# Autodesk Inventor assembly: mascon-new
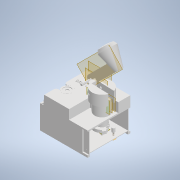
[picture p0: Inventor's stored thumbnail of the model, 180x180]
Saved by Autodesk Inventor 2022 (Build 260153000, 153)
## iProperties
Created: 2021-04-28
Part Number: mascon-new
Document SubType Name: Assembly
Designer: ben
Author: ben
## iProperties of the stored document Pin2.ipt
Created: 2022-01-01
Part Number: Pin2
Material: Steel
Document SubType Name: Modeling
Designer: teh18
Density: 7.85 g/cm^3
Appearance: Default
Author: teh18
## iProperties of the stored document ScrewBase.ipt
Created: 2022-01-01
Part Number: ScrewBase
Material: Steel
Document SubType Name: Modeling
Designer: teh18
Density: 7.85 g/cm^3
Appearance: Default
Author: teh18
## iProperties of the stored document Pin3.ipt
Created: 2022-01-01
Part Number: Pin3
Material: Steel
Document SubType Name: Modeling
Designer: teh18
Density: 7.85 g/cm^3
Appearance: Default
Author: teh18
## iProperties of the stored document Board.ipt
Created: 2022-01-01
Part Number: Board
Material: Steel
Document SubType Name: Modeling
Designer: teh18
Density: 7.85 g/cm^3
Appearance: Default
Author: teh18
## iProperties of the stored document Casing.ipt
Created: 2022-01-01
Part Number: Casing
Material: Steel
Document SubType Name: Modeling
Designer: teh18
Density: 7.85 g/cm^3
Appearance: Default
Author: teh18
## iProperties of the stored document Pin1.ipt
Created: 2022-01-01
Part Number: Pin1
Material: Steel
Document SubType Name: Modeling
Designer: teh18
Density: 7.85 g/cm^3
Appearance: Default
Author: teh18
## iProperties of the stored document PotentiometerB10K.iam
Created: 2020-08-30
Part Number: PotentiometerB10K
Document SubType Name: Assembly
Designer: teh18
Title: D:/OneDrive/Projetos/Yoke FS/V4/PotentiometerToGrabCad/PotentiometerB10K.step
Sending System: Autodesk Translation Framework v9.3.0.1241
Preprocessor: ST-DEVELOPER v18.1
## iProperties of the stored document Shaft.ipt
Created: 2022-01-01
Part Number: Shaft
Material: Steel
Document SubType Name: Modeling
Designer: teh18
Density: 7.85 g/cm^3
Appearance: Default
Author: teh18
## Documents named in this file (20)
- **C:\Users\teh18\Documents\GitHub\r68-bve-mascon\mascon-new.iam*LocalDocs*xAaaaahdaAaaaaaaaAaaaakmpVc*Pin2.ipt
- **C:\Users\teh18\Documents\GitHub\r68-bve-mascon\mascon-new.iam*LocalDocs*xAaaaafdaAaaaaaaaAaaaabwyVb*ScrewBase.ipt
- **C:\Users\teh18\Documents\GitHub\r68-bve-mascon\mascon-new.iam*LocalDocs*xAaaaaccaAaaaaaaaAaaaacpb2b*Pin3.ipt
- **C:\Users\teh18\Documents\GitHub\r68-bve-mascon\mascon-new.iam*LocalDocs*xAaaaagaaAaaaaaaaAaaaqhofGg*Board.ipt
- **C:\Users\teh18\Documents\GitHub\r68-bve-mascon\mascon-new.iam*LocalDocs*xAaaaqjcaAaaaaaaaAaaaat2iJf*Casing.ipt
- **C:\Users\teh18\Documents\GitHub\r68-bve-mascon\mascon-new.iam*LocalDocs*xAaaaqfaaAaaaaaaaAaaaaacoKh*Pin1.ipt
- **C:\Users\teh18\Documents\GitHub\r68-bve-mascon\mascon-new.iam*LocalDocs*xAaaaqhaaAaaaaaaaAaaaaeywJf*PotentiometerB10K.iam
- **C:\Users\teh18\Documents\GitHub\r68-bve-mascon\mascon-new.iam*LocalDocs*xAaaaqrbaAaaaaaaaAaaaalw5Ad*Shaft.ipt
- C:\Users\teh18\Documents\GitHub\r68-bve-mascon\mascon-new.iam
- C:\Users\teh18\Documents\GitHub\r68-bve-mascon\handle\handle.iam
- C:\Users\teh18\Documents\GitHub\r68-bve-mascon\shell\shell.iam
- C:\Users\teh18\Documents\GitHub\r68-bve-mascon\handle_holder.ipt
- C:\Users\teh18\Documents\GitHub\r68-bve-mascon\Reverser.ipt
- C:\Users\teh18\Documents\GitHub\r68-bve-mascon\handle-base\handle_base.iam
- C:\Users\teh18\Documents\GitHub\r68-bve-mascon\handle_base2.ipt
- C:\Users\teh18\Documents\GitHub\r68-bve-mascon\handle-base\SpringRod.ipt
- C:\Users\teh18\Documents\GitHub\r68-bve-mascon\handle-base\PotAttachmentB10L.ipt
- C:\Users\teh18\Documents\GitHub\r68-bve-mascon\handle-base\PotAttachmentB10R.ipt
- C:\Users\teh18\Documents\GitHub\r68-bve-mascon\mascon-new\Design Accelerator\Spur Gears1.iam
- C:\Users\teh18\Documents\GitHub\r68-bve-mascon\potentiometer-b10k-1.snapshot.2\PotentiometerB10K.step
## Components (12 placed, 11 different names)
1. shell:1 [sub-assembly] — Flush:4, Mate:29, Mate:30, Mate:37, Mate:38
2. handle_holder:1
3. Reverser:1 — Flush:4
4. handle:1 [sub-assembly]
5. handle_base:1 [sub-assembly] — Mate:29, Mate:30, Mate:34, Mate:35, Mate:36
6. handle_base2:1 — Mate:34, Mate:35, Mate:36, Mate:39, Mate:40
7. SpringRod:1
8. PotentiometerB10K:1 [sub-assembly] — Mate:37, Mate:38, Mate:41, Mate:42
9. PotentiometerB10K:2 [sub-assembly]
10. PotAttachmentB10L:1 — Mate:39, Mate:40
11. PotAttachmentB10R:1 — Mate:41, Mate:42
12. Spur Gears:1 [sub-assembly]
## Relationships (12: Mate 11, Flush 1)
- Flush:4: shell:1 ↔ Reverser:1
- Mate:29: shell:1 ↔ handle_base:1
- Mate:30: shell:1 ↔ handle_base:1
- Mate:34: handle_base:1 ↔ handle_base2:1
- Mate:35: handle_base:1 ↔ handle_base2:1
- Mate:36: handle_base:1 ↔ handle_base2:1
- Mate:37: shell:1 ↔ PotentiometerB10K:1
- Mate:38: shell:1 ↔ PotentiometerB10K:1
- Mate:39: handle_base2:1 ↔ PotAttachmentB10L:1
- Mate:40: handle_base2:1 ↔ PotAttachmentB10L:1
- Mate:41: PotentiometerB10K:1 ↔ PotAttachmentB10R:1
- Mate:42: PotentiometerB10K:1 ↔ PotAttachmentB10R:1
